# Autodesk Inventor assembly: nut_and_holder
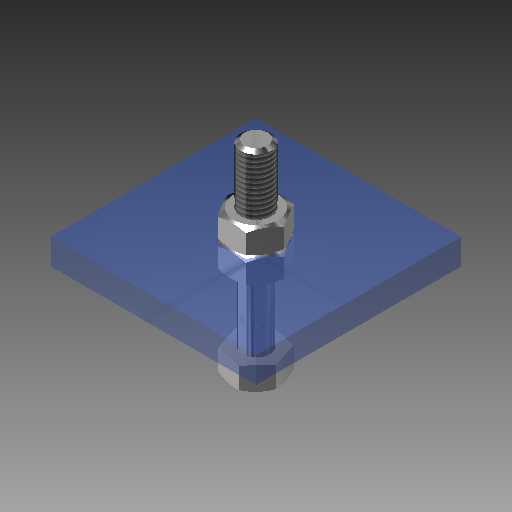
[picture p0: Inventor's stored thumbnail of the model, 512x512]
Saved by Autodesk Inventor 2018.1 (Build 221171000, 171)
## iProperties
Created: 2017-07-29
Part Number: nut_and_holder
Document SubType Name: Assembly
Designer: Tom
Mass: 196.193 g
Surface Area: 223.195 cm^2
Volume: 75.0099 cm^3
Density: 2.61556 g/cm^3
Author: Tom
## Documents named in this file (4)
- \\Mac\Dropbox\2015-2016\Bachelorproef\Inventor\Etstank_v2\platform_nut_holder_assembly.iam
- \\Mac\Dropbox\2015-2016\Bachelorproef\Inventor\Etstank_v2\platform_nut holder.ipt
- \\Mac\Home\Documents\Inventor\Content Center Files\R2018\en-US\DIN 934\DIN 934 - M12 x 1,75.ipt
- \\Mac\Home\Documents\Inventor\Content Center Files\R2018\en-US\ANSI B 18.6.7 M IFI 513(5)\ANSI B 18.6.7 M _ IFI 513 - M12 x 1,75 x 70(3).ipt
## Components (4 placed, 3 different names)
1. DIN 934 - replaced by DIN EN 24032/28673/28674 M12:3 — Mate:1, Flush:1, Mate:2, Mate:4, Mate:7
2. platform_nut holder:1 — Mate:1, Flush:1, Mate:2, Mate:3, Mate:5
3. Trimmed Hex Head Machine Screw - Metric M12 x 1,75 x 70:1 — Mate:4, Mate:5, Mate:6
4. DIN 934 - replaced by DIN EN 24032/28673/28674 M12:4 — Mate:6, Mate:7
## Relationships (8: Mate 7, Flush 1)
- Mate:1: DIN 934 - replaced by DIN EN 24032/28673/28674 M12:3 ↔ platform_nut holder:1
- Flush:1: DIN 934 - replaced by DIN EN 24032/28673/28674 M12:3 ↔ platform_nut holder:1
- Mate:2: DIN 934 - replaced by DIN EN 24032/28673/28674 M12:3 ↔ platform_nut holder:1
- Mate:3: platform_nut holder:1
- Mate:4: DIN 934 - replaced by DIN EN 24032/28673/28674 M12:3 ↔ Trimmed Hex Head Machine Screw - Metric M12 x 1,75 x 70:1
- Mate:5 (27 mm): platform_nut holder:1 ↔ Trimmed Hex Head Machine Screw - Metric M12 x 1,75 x 70:1
- Mate:6: Trimmed Hex Head Machine Screw - Metric M12 x 1,75 x 70:1 ↔ DIN 934 - replaced by DIN EN 24032/28673/28674 M12:4
- Mate:7: DIN 934 - replaced by DIN EN 24032/28673/28674 M12:3 ↔ DIN 934 - replaced by DIN EN 24032/28673/28674 M12:4
